# Autodesk Inventor assembly: PIT
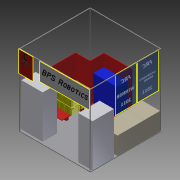
[picture p0: Inventor's stored thumbnail of the model, 180x180]
Saved by Autodesk Inventor 2014 (Build 180170000, 170)
## iProperties
Created: 2015-04-10
Part Number: PIT
Document SubType Name: Assembly
Designer: Gus
Author: Gus
## Documents named in this file (16)
- C:\Users\Public\Documents\Autodesk\Vault Basic 2014\Samples\Inventor 2014\Padlock\Designs\PIT.iam
- C:\Users\Public\Documents\Autodesk\Vault Basic 2014\Samples\Inventor 2014\Padlock\Designs\parts\pit_floor.ipt
- C:\Users\Public\Documents\Autodesk\Vault Basic 2014\Samples\Inventor 2014\Padlock\Designs\parts\crate.ipt
- C:\Users\Public\Documents\Autodesk\Vault Basic 2014\Samples\Inventor 2014\Padlock\Designs\parts\YELLOW_TOTE.ipt
- C:\Users\Public\Documents\Autodesk\Vault Basic 2014\Samples\Inventor 2014\Padlock\Designs\parts\YELLOW_TOTEASM_ASM.iam
- YELLOW_TOTEASM_ASM.ipt
- C:\Users\Public\Documents\Autodesk\Vault Basic 2014\Samples\Inventor 2014\Padlock\Designs\parts\RECYCLING_BIN_ASM.iam
- RECYCLING_BIN_ASM.ipt
- C:\Users\Public\Documents\Autodesk\Vault Basic 2014\Samples\Inventor 2014\Padlock\Designs\parts\tool  chest.ipt
- C:\Users\Public\Documents\Autodesk\Vault Basic 2014\Samples\Inventor 2014\Padlock\Designs\parts\shelves.ipt
- C:\Users\Public\Documents\Autodesk\Vault Basic 2014\Samples\Inventor 2014\Padlock\Designs\parts\table.ipt
- C:\Users\Public\Documents\Autodesk\Vault Basic 2014\Samples\Inventor 2014\Padlock\Designs\parts\banner1.ipt
- C:\Users\Public\Documents\Autodesk\Vault Basic 2014\Samples\Inventor 2014\Padlock\Designs\parts\banner2.ipt
- C:\Users\Public\Documents\Autodesk\Vault Basic 2014\Samples\Inventor 2014\Padlock\Designs\parts\canopy.ipt
- C:\Users\Public\Documents\Autodesk\Vault Basic 2014\Samples\Inventor 2014\Padlock\Designs\parts\Winner Banner.ipt
- C:\Users\Public\Documents\Autodesk\Vault Basic 2014\Samples\Inventor 2014\Padlock\Designs\parts\Chairmans Award Banner.ipt
## Components (16 placed, 13 different names)
1. pit_floor:1 — Mate:1, Mate:6, Mate:7
2. crate:1 — Mate:1, Mate:2, Mate:4, Mate:5
3. YELLOW_TOTE:1 — Mate:3
4. YELLOW_TOTE:2 — Mate:2, Mate:3
5. RECYCLING_BIN_ASM:1 [sub-assembly] — Mate:4
6. tool  chest:1 — Mate:5
7. shelves:1 — Mate:6
8. shelves:2 — Mate:7
9. table:1
10. banner1:1
11. banner2:1
12. YELLOW_TOTEASM_ASM:2 [sub-assembly]
13. YELLOW_TOTEASM_ASM:3 [sub-assembly]
14. canopy:1
15. Winner Banner:1
16. Chairmans Award Banner:1
## Relationships (7: Mate 7)
- Mate:1: pit_floor:1 ↔ crate:1
- Mate:2: crate:1 ↔ YELLOW_TOTE:2
- Mate:3: YELLOW_TOTE:1 ↔ YELLOW_TOTE:2
- Mate:4: crate:1 ↔ RECYCLING_BIN_ASM:1
- Mate:5: crate:1 ↔ tool  chest:1
- Mate:6: pit_floor:1 ↔ shelves:1
- Mate:7: pit_floor:1 ↔ shelves:2
